# Autodesk Inventor assembly: am-3312a_Gear Intake Kit Gear Config
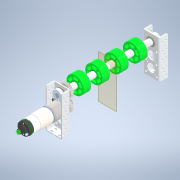
[picture p0: Inventor's stored thumbnail of the model, 180x180]
Saved by Autodesk Inventor 2020.2 (Build 242310000, 310)
## iProperties
Created: 2018-12-20
Part Number: am-3312a_Gear Intake Kit Gear Config
Description: STEP AP214
Document SubType Name: Assembly
Designer: robst
Sending System: SolidWorks 2018
Preprocessor: SwSTEP 2.0
Title: am-3312a_Gear Intake Kit Gear Config.STEP
Revision Number: ANY
## Documents named in this file (15)
- C:\git\CAD-Development\robSteele\2020CompetitionRobot\am-3312a_Gear Intake Kit Gear Config.iam
- C:\git\CAD-Development\robSteele\2020LongRobotBase\rev3plate.ipt
- C:\git\CAD-Development\robSteele\2020LongRobotBase\FR8ZZ Hex Bearing.ipt
- C:\git\CAD-Development\robSteele\2020LongRobotBase\10-32x03125 - Mcm 91251A337_91251A337.ipt
- C:\git\CAD-Development\robSteele\2020LongRobotBase\flat washer type a wide_ai_Preferred Wide FW 0.25.ipt
- C:\git\CAD-Development\robSteele\2020LongRobotBase\500 Hex main axle.ipt
- C:\git\CAD-Development\robSteele\2020LongRobotBase\am-3654 PG27 500 hex+Motor+Encoder.iam
- C:\git\CAD-Development\robSteele\2020LongRobotBase\Hex Collar 500.ipt
- C:\git\CAD-Development\robSteele\2020LongRobotBase\am-3948-125 500H x 125IN Spacer.ipt
- C:\git\CAD-Development\robSteele\2020LongRobotBase\1.475in Hex Spacer Extrusion.ipt
- C:\git\CAD-Development\robSteele\2020LongRobotBase\BHCS 10-32 x 0.625 patch_92360A219.ipt
- C:\git\CAD-Development\robSteele\2020LongRobotBase\32T 20DP 500hex 375 FW.ipt
- C:\git\CAD-Development\robSteele\2020LongRobotBase\am-3948-250 500H x 250IN Spacer.ipt
- C:\git\CAD-Development\robSteele\2020LongRobotBase\.906in Hex Spacer Extrusion.ipt
- C:\git\CAD-Development\robSteele\2020LongRobotBase\am-3949 2.25N OverMolded 500Hex Compliant Wheel V6.iam
## Components (30 placed, 30 different names)
1. rev3plate_1 — Flush:1
2. FR8ZZ Hex Bearing_2
3. 10-32x03125 - Mcm 91251A337_91251A337_3
4. flat washer type a wide_ai_Preferred Wide FW 0.25_4
5. 500 Hex main axle_5
6. rev3plate_6 — Flush:2
7. FR8ZZ Hex Bearing_7
8. am-3654 PG27 500 hex+Motor+Encoder_8 [sub-assembly]
9. Hex Collar 500_9
10. Hex Collar 500_10
11. am-3948-125 500H x 125IN Spacer_11
12. 1.475in Hex Spacer Extrusion_12
13. 1.475in Hex Spacer Extrusion_13
14. 1.475in Hex Spacer Extrusion_14
15. 1.475in Hex Spacer Extrusion_15
16. am-3948-125 500H x 125IN Spacer_16
17. BHCS 10-32 x 0.625 patch_92360A219_17
18. BHCS 10-32 x 0.625 patch_92360A219_18
19. BHCS 10-32 x 0.625 patch_92360A219_19
20. BHCS 10-32 x 0.625 patch_92360A219_20
21. 32T 20DP 500hex 375 FW_21
22. am-3948-250 500H x 250IN Spacer_22
23. am-3948-250 500H x 250IN Spacer_23
24. 32T 20DP 500hex 375 FW_24
25. am-3948-125 500H x 125IN Spacer_25
26. .906in Hex Spacer Extrusion_26
27. am-3949 2.25N OverMolded 500Hex Compliant Wheel V6_27 [sub-assembly]
28. am-3949 2.25N OverMolded 500Hex Compliant Wheel V6_28 [sub-assembly]
29. am-3949 2.25N OverMolded 500Hex Compliant Wheel V6_29 [sub-assembly]
30. am-3949 2.25N OverMolded 500Hex Compliant Wheel V6_30 [sub-assembly]
## Relationships (2: Flush 2)
- Flush:1 (148.412 mm): rev3plate_1
- Flush:2 (146.4125 mm): rev3plate_6
